# Autodesk Inventor assembly: Assembly2
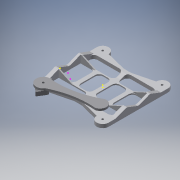
[picture p0: Inventor's stored thumbnail of the model, 180x180]
Saved by Autodesk Inventor 2016 (Build 200138000, 138)
## iProperties
Created: 2016-01-12
Part Number: Assembly2
Document SubType Name: Assembly
Designer: cemer
Author: cemer
## Documents named in this file (3)
- C:\Users\cemer\Desktop\Assembly2.iam
- C:\Users\cemer\Desktop\Part1.ipt
- C:\Users\cemer\Desktop\Part2.ipt
## Components (2 placed, 2 different names)
1. Part1:1 — Rotational:1
2. Part2:1 — Rotational:1
## Relationships (1: RevoluteJoint 1)
- Rotational:1 [RevoluteJoint]: Part1:1 ↔ Part2:1
